# Autodesk Inventor assembly: 試作品1号コピー
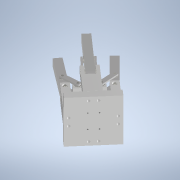
[picture p0: Inventor's stored thumbnail of the model, 180x180]
Saved by Autodesk Inventor 2021 (Build 250183000, 183)
## iProperties
Created: 2021-10-09
Part Number: 試作品1号コピー
Document SubType Name: Assembly
Designer: ryusei
Author: ryusei
## Documents named in this file (13)
- C:\Users\ryusei\Documents\Inventor\robot_design3\試作品1号\試作品1号コピー.iam
- C:\Users\ryusei\Documents\Inventor\robot_design3\試作品1号\土台.ipt
- C:\Users\ryusei\Documents\Inventor\robot_design3\試作品1号\アーム支え.ipt
- C:\Users\ryusei\Documents\Inventor\robot_design3\試作品1号\MF63ZZ_ベアリング.ipt
- C:\Users\ryusei\Documents\Inventor\robot_design3\試作品1号\ステンレス平行ピンΦ3h7_20.ipt
- C:\Users\ryusei\Documents\Inventor\robot_design3\試作品1号\シリンダ固定.ipt
- C:\Users\ryusei\Documents\Inventor\robot_design3\試作品1号\シリンダ先端パーツ.ipt
- C:\Users\ryusei\Documents\Inventor\robot_design3\試作品1号\MBDA6×15_シリンダコガネイ\伸びるやつ１.ipt
- C:\Users\ryusei\Documents\Inventor\robot_design3\試作品1号\MBDA6×15_シリンダコガネイ\伸びるやつ2.ipt
- C:\Users\ryusei\Documents\Inventor\robot_design3\試作品1号\MBDA6×15_シリンダコガネイ\本体.ipt
- C:\Users\ryusei\Documents\Inventor\robot_design3\試作品1号\アーム10×10×60.ipt
- C:\Users\ryusei\Documents\Inventor\robot_design3\試作品1号\ステンレス平行ピンΦ3h7_16.ipt
- C:\Users\ryusei\Documents\Inventor\robot_design3\試作品1号\リンク26×6×2.ipt
## Components (59 placed, 12 different names)
1. 土台:1
2. アーム支え:1
3. アーム支え:2
4. アーム支え:3
5. アーム支え:4
6. MF63ZZ_ベアリング:1
7. MF63ZZ_ベアリング:2
8. MF63ZZ_ベアリング:3
9. MF63ZZ_ベアリング:4
10. MF63ZZ_ベアリング:5
11. MF63ZZ_ベアリング:6
12. MF63ZZ_ベアリング:7
13. MF63ZZ_ベアリング:8
14. ステンレス平行ピンΦ3h7_20:1
15. ステンレス平行ピンΦ3h7_20:2
16. ステンレス平行ピンΦ3h7_20:3
17. シリンダ固定:1
18. シリンダ固定:2
19. アーム10×10×60:1
20. アーム10×10×60:2
21. アーム10×10×60:3
22. アーム10×10×60:4
23. MF63ZZ_ベアリング:9
24. MF63ZZ_ベアリング:10
25. MF63ZZ_ベアリング:11
26. MF63ZZ_ベアリング:12
27. MF63ZZ_ベアリング:13
28. MF63ZZ_ベアリング:14
29. MF63ZZ_ベアリング:15
30. MF63ZZ_ベアリング:16
31. ステンレス平行ピンΦ3h7_16:1
32. ステンレス平行ピンΦ3h7_16:2
33. ステンレス平行ピンΦ3h7_16:3
34. ステンレス平行ピンΦ3h7_16:4
35. シリンダ先端パーツ:1
36. 伸びるやつ１:1
37. 伸びるやつ2:1
38. 本体:1
39. MF63ZZ_ベアリング:17
40. MF63ZZ_ベアリング:18
41. MF63ZZ_ベアリング:19
42. MF63ZZ_ベアリング:20
43. MF63ZZ_ベアリング:21
44. MF63ZZ_ベアリング:22
45. MF63ZZ_ベアリング:23
46. MF63ZZ_ベアリング:24
47. ステンレス平行ピンΦ3h7_16:5
48. ステンレス平行ピンΦ3h7_16:6
49. ステンレス平行ピンΦ3h7_16:7
50. ステンレス平行ピンΦ3h7_16:8
51. ステンレス平行ピンΦ3h7_20:4
52. リンク26×6×2:1
53. リンク26×6×2:2
54. リンク26×6×2:3
55. リンク26×6×2:4
56. リンク26×6×2:5
57. リンク26×6×2:6
58. リンク26×6×2:7
59. リンク26×6×2:8
## Relationships (92: Insert 74, Mate 17, Angle 1)
- [Insert]: 土台:1 ↔ アーム支え:4
- [Insert]: 土台:1 ↔ アーム支え:4
- [Insert]: 土台:1 ↔ アーム支え:3
- [Insert]: 土台:1 ↔ アーム支え:3
- [Insert]: 土台:1 ↔ アーム支え:1
- [Insert]: 土台:1 ↔ アーム支え:1
- [Insert]: 土台:1 ↔ アーム支え:2
- [Insert]: 土台:1 ↔ アーム支え:2
- [Insert]: アーム支え:1 ↔ MF63ZZ_ベアリング:8
- [Insert]: アーム支え:1 ↔ MF63ZZ_ベアリング:3
- [Insert]: アーム支え:2 ↔ MF63ZZ_ベアリング:6
- [Insert]: アーム支え:2 ↔ MF63ZZ_ベアリング:4
- [Insert]: アーム支え:3 ↔ MF63ZZ_ベアリング:2
- [Insert]: アーム支え:3 ↔ MF63ZZ_ベアリング:7
- [Insert]: アーム支え:4 ↔ MF63ZZ_ベアリング:1
- [Insert]: アーム支え:4 ↔ MF63ZZ_ベアリング:5
- [Mate]: MF63ZZ_ベアリング:8 ↔ ステンレス平行ピンΦ3h7_20:3
- [Mate]: MF63ZZ_ベアリング:2 ↔ ステンレス平行ピンΦ3h7_20:2
- [Mate]: MF63ZZ_ベアリング:6 ↔ ステンレス平行ピンΦ3h7_20:1
- [Insert]: 土台:1 ↔ シリンダ固定:1
- [Insert]: 土台:1 ↔ シリンダ固定:1
- [Insert]: 土台:1 ↔ シリンダ固定:2
- [Insert]: 土台:1 ↔ シリンダ固定:2
- [Mate]: ステンレス平行ピンΦ3h7_20:2 ↔ アーム10×10×60:3
- [Mate]: ステンレス平行ピンΦ3h7_20:3 ↔ アーム10×10×60:2
- [Mate]: ステンレス平行ピンΦ3h7_20:1 ↔ アーム10×10×60:1
- [Insert]: アーム10×10×60:2 ↔ MF63ZZ_ベアリング:16
- [Insert]: アーム10×10×60:2 ↔ MF63ZZ_ベアリング:15
- [Insert]: アーム10×10×60:4 ↔ MF63ZZ_ベアリング:11
- [Insert]: アーム10×10×60:4 ↔ MF63ZZ_ベアリング:12
- [Insert]: アーム10×10×60:3 ↔ MF63ZZ_ベアリング:13
- [Insert]: アーム10×10×60:3 ↔ MF63ZZ_ベアリング:14
- [Insert]: アーム10×10×60:1 ↔ MF63ZZ_ベアリング:9
- [Insert]: アーム10×10×60:1 ↔ MF63ZZ_ベアリング:10
- [Mate]: MF63ZZ_ベアリング:11 ↔ ステンレス平行ピンΦ3h7_16:3
- [Mate]: MF63ZZ_ベアリング:13 ↔ ステンレス平行ピンΦ3h7_16:4
- [Mate]: MF63ZZ_ベアリング:16 ↔ ステンレス平行ピンΦ3h7_16:2
- [Mate]: MF63ZZ_ベアリング:9 ↔ ステンレス平行ピンΦ3h7_16:1
- [Insert]: 伸びるやつ１:1 ↔ 伸びるやつ2:1
- [Mate]: 伸びるやつ１:1 ↔ 本体:1
- [Insert]: シリンダ先端パーツ:1 ↔ 伸びるやつ１:1
- [Insert]: シリンダ固定:2 ↔ 本体:1
- [Insert]: シリンダ固定:2 ↔ 本体:1
- [Angle] (0 deg): 土台:1 ↔ シリンダ先端パーツ:1
- [Insert]: シリンダ先端パーツ:1 ↔ MF63ZZ_ベアリング:20
- [Insert]: シリンダ先端パーツ:1 ↔ MF63ZZ_ベアリング:19
- [Insert]: シリンダ先端パーツ:1 ↔ MF63ZZ_ベアリング:18
- [Insert]: シリンダ先端パーツ:1 ↔ MF63ZZ_ベアリング:17
- [Insert]: シリンダ先端パーツ:1 ↔ MF63ZZ_ベアリング:21
- [Insert]: シリンダ先端パーツ:1 ↔ MF63ZZ_ベアリング:22
- [Insert]: シリンダ先端パーツ:1 ↔ MF63ZZ_ベアリング:23
- [Insert]: シリンダ先端パーツ:1 ↔ MF63ZZ_ベアリング:24
- [Mate]: MF63ZZ_ベアリング:17 ↔ ステンレス平行ピンΦ3h7_16:7
- [Mate]: MF63ZZ_ベアリング:21 ↔ ステンレス平行ピンΦ3h7_16:6
- [Mate]: MF63ZZ_ベアリング:20 ↔ ステンレス平行ピンΦ3h7_16:5
- [Mate]: MF63ZZ_ベアリング:23 ↔ ステンレス平行ピンΦ3h7_16:8
- [Insert]: 土台:1 ↔ アーム支え:2
- [Insert]: 土台:1 ↔ アーム支え:2
- [Insert]: 土台:1 ↔ アーム支え:3
- [Insert]: 土台:1 ↔ アーム支え:3
- [Insert]: 土台:1 ↔ アーム支え:2
- [Insert]: 土台:1 ↔ アーム支え:2
- [Insert]: 土台:1 ↔ アーム支え:1
- [Insert]: 土台:1 ↔ アーム支え:1
- [Insert]: 土台:1 ↔ アーム支え:4
- [Insert]: 土台:1 ↔ アーム支え:4
- [Insert]: 土台:1 ↔ アーム支え:2
- [Insert]: 土台:1 ↔ アーム支え:2
- [Insert]: 土台:1 ↔ アーム支え:3
- [Insert]: 土台:1 ↔ アーム支え:3
- [Insert]: 土台:1 ↔ アーム支え:4
- [Insert]: 土台:1 ↔ アーム支え:4
- [Insert]: 土台:1 ↔ アーム支え:1
- [Insert]: 土台:1 ↔ アーム支え:1
- [Mate]: MF63ZZ_ベアリング:5 ↔ ステンレス平行ピンΦ3h7_20:4
- [Mate]: アーム10×10×60:4 ↔ ステンレス平行ピンΦ3h7_20:4
- [Insert]: ステンレス平行ピンΦ3h7_16:1 ↔ リンク26×6×2:8
- [Insert]: ステンレス平行ピンΦ3h7_16:7 ↔ リンク26×6×2:8
- [Insert]: ステンレス平行ピンΦ3h7_16:6 ↔ リンク26×6×2:7
- [Insert]: ステンレス平行ピンΦ3h7_16:4 ↔ リンク26×6×2:7
- [Insert]: ステンレス平行ピンΦ3h7_16:6 ↔ リンク26×6×2:6
- [Insert]: ステンレス平行ピンΦ3h7_16:4 ↔ リンク26×6×2:6
- [Insert]: ステンレス平行ピンΦ3h7_16:8 ↔ リンク26×6×2:1
- [Insert]: ステンレス平行ピンΦ3h7_16:3 ↔ リンク26×6×2:1
- [Insert]: ステンレス平行ピンΦ3h7_16:8 ↔ リンク26×6×2:5
- [Insert]: ステンレス平行ピンΦ3h7_16:3 ↔ リンク26×6×2:5
- [Insert]: ステンレス平行ピンΦ3h7_16:2 ↔ リンク26×6×2:4
- [Insert]: ステンレス平行ピンΦ3h7_16:5 ↔ リンク26×6×2:4
- [Insert]: ステンレス平行ピンΦ3h7_16:7 ↔ リンク26×6×2:3
- [Insert]: ステンレス平行ピンΦ3h7_16:1 ↔ リンク26×6×2:3
- [Insert]: ステンレス平行ピンΦ3h7_16:5 ↔ リンク26×6×2:2
- [Insert]: ステンレス平行ピンΦ3h7_16:2 ↔ リンク26×6×2:2
